# Autodesk Inventor assembly: Port_Rudder
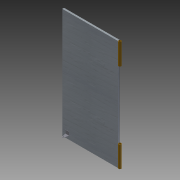
[picture p0: Inventor's stored thumbnail of the model, 180x180]
Saved by Autodesk Inventor 2011 SP1 (Build 150282100, 282)
## iProperties
Created: 2011-06-11
Part Number: Port_Rudder
Document SubType Name: Assembly
Designer: Andrew G. Meyer
Mass: 46.714 g
Surface Area: 333.539 cm^2
Volume: 46.714 cm^3
Density: 1 g/cm^3
Author: Andrew G. Meyer
## Documents named in this file (3)
- C:\Users\Andrew G. Meyer\Documents\Inventor\Hovercraft\Port_Rudder.iam
- C:\Users\Andrew G. Meyer\Documents\Inventor\Hovercraft\Rudder_Base.iam
- C:\Users\Andrew G. Meyer\Documents\Inventor\Hovercraft\Control_Horn.ipt
## Components (2 placed, 2 different names)
1. Rudder_Base:1 [sub-assembly] — Mate:1, Flush:1, Flush:2
2. Control_Horn:1 — Mate:1, Flush:1, Flush:2
## Relationships (3: Flush 2, Mate 1)
- Mate:1: Rudder_Base:1 ↔ Control_Horn:1
- Flush:1 (6.35 mm): Rudder_Base:1 ↔ Control_Horn:1
- Flush:2 (6.35 mm): Rudder_Base:1 ↔ Control_Horn:1
